# Autodesk Inventor assembly: body
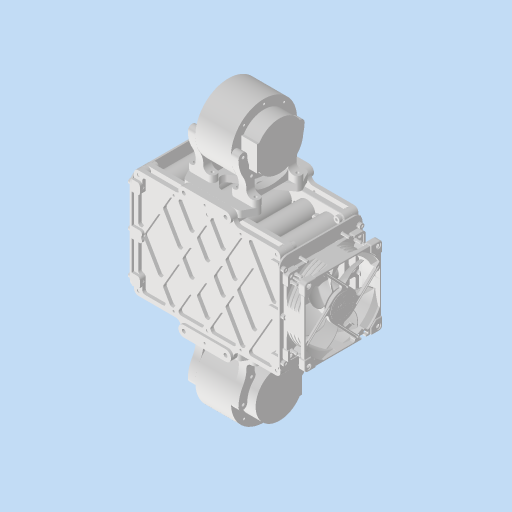
[picture p0: Inventor's stored thumbnail of the model, 512x512]
Saved by Autodesk Inventor 2023 (Build 270158000, 158)
## iProperties
Created: 2026-05-26
Part Number: body
Document SubType Name: Assembly
Designer: Nathann
Author: Nathann
## iProperties of the stored document MemberDocs/xQqurx3pxBk00kwhm3pl5gy5wAf
Created: 2026-05-26
Part Number: body
Document SubType Name: Assembly
Designer: Nathann
Author: Nathann
## Documents named in this file (6)
- C:\Users\Nathann\OneDrive\ClawdDrive\Objet3D\RunningRobot\PartURDF\body.iam
- C:\Users\Nathann\OneDrive\ClawdDrive\Objet3D\RunningRobot\testChassis.iam
- C:\Users\Nathann\OneDrive\ClawdDrive\Objet3D\RunningRobot\testChassis Connector.ipt
- C:\Users\Nathann\OneDrive\ClawdDrive\Objet3D\RunningRobot\testHip Hinge Base.ipt
- C:\Users\Nathann\OneDrive\ClawdDrive\Objet3D\RunningRobot\testHip Hinge Base 2.ipt
- C:\Users\Nathann\OneDrive\ClawdDrive\Objet3D\RunningRobot\testAK-60 Phantom_Défaut_1.iam
## Components (9 placed, 5 different names)
1. testChassis:1 [sub-assembly] — Mate:1, Mate:2, Flush:1, Insert:1, Insert:2, Insert:9, Insert:10
2. testChassis Connector:1 — Insert:1, Insert:2, Insert:3, Insert:4, Insert:5, Insert:6
3. testHip Hinge Base:1 — Insert:3, Insert:4, Insert:7, Insert:8
4. testHip Hinge Base 2:1 — Insert:5, Insert:6
5. testAK-60 Phantom_Défaut_1:1 [sub-assembly] — Insert:7, Insert:8
6. testChassis Connector:2 — Insert:9, Insert:10, Insert:11, Insert:12, Insert:13, Insert:14
7. testHip Hinge Base:2 — Insert:13, Insert:14, Insert:15, Insert:16
8. testHip Hinge Base 2:2 — Insert:11, Insert:12
9. testAK-60 Phantom_Défaut_1:2 [sub-assembly] — Insert:15, Insert:16
## Relationships (19: Insert 16, Mate 2, Flush 1)
- Mate:1: testChassis:1
- Mate:2: testChassis:1
- Flush:1: testChassis:1
- Insert:1: testChassis:1 ↔ testChassis Connector:1
- Insert:2: testChassis:1 ↔ testChassis Connector:1
- Insert:3: testChassis Connector:1 ↔ testHip Hinge Base:1
- Insert:4: testChassis Connector:1 ↔ testHip Hinge Base:1
- Insert:5: testChassis Connector:1 ↔ testHip Hinge Base 2:1
- Insert:6: testChassis Connector:1 ↔ testHip Hinge Base 2:1
- Insert:7: testHip Hinge Base:1 ↔ testAK-60 Phantom_Défaut_1:1
- Insert:8: testHip Hinge Base:1 ↔ testAK-60 Phantom_Défaut_1:1
- Insert:9: testChassis:1 ↔ testChassis Connector:2
- Insert:10: testChassis:1 ↔ testChassis Connector:2
- Insert:11: testChassis Connector:2 ↔ testHip Hinge Base 2:2
- Insert:12: testChassis Connector:2 ↔ testHip Hinge Base 2:2
- Insert:13: testChassis Connector:2 ↔ testHip Hinge Base:2
- Insert:14: testChassis Connector:2 ↔ testHip Hinge Base:2
- Insert:15: testHip Hinge Base:2 ↔ testAK-60 Phantom_Défaut_1:2
- Insert:16: testHip Hinge Base:2 ↔ testAK-60 Phantom_Défaut_1:2
